# Autodesk Inventor assembly: 4in Omni Duallie
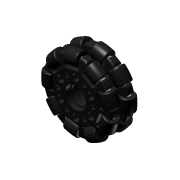
[picture p0: Inventor's stored thumbnail of the model, 180x180]
Saved by Autodesk Inventor 2011 (Build 150239000, 239)
## iProperties
Created: 2011-07-02
Part Number: 4in Omni Duallie
Document SubType Name: Assembly
Designer: Dan Niemitalo
Mass: 317.515 g
Surface Area: 1028.24 cm^2
Volume: 193.792 cm^3
Translation Standard: STEP AP203
FileName: //Amserv/amserver/AndyMark/Products/4 inch omni wheel/4 inch omni wheel dualie w 500 bearings.stp
PreProcessor: Unknown
PostProcessor: Build: 282, Release: 2011 SP1 - Date: Thu 08/05/2010
Sent Units: millimeter
Uncertainty: 0.001
Author: Dan Niemitalo
## Documents named in this file (3)
- H:\Nemo\Documents\Robotics\COTS Parts\Wheels\4in Omni Dualie.iam
- H:\Nemo\Documents\Robotics\Wheels and Sprockets\4 inch omni wheel no bearings.iam
- H:\Nemo\Documents\Robotics\COTS Parts\Sprockets\250 sprocket spacer.ipt
## Components (3 placed, 2 different names)
1. 250 sprocket spacer:1 — Mate:1, Mate:2, Mate:3, Mate:5, Mate:6, Mate:7
2. 4 inch omni wheel no bearings:1 [sub-assembly] — Mate:2, Mate:6, Mate:7
3. 4 inch omni wheel no bearings:2 [sub-assembly] — Mate:1, Mate:3, Mate:5
## Relationships (6: Mate 6)
- Mate:1: 250 sprocket spacer:1 ↔ 4 inch omni wheel no bearings:2
- Mate:2: 250 sprocket spacer:1 ↔ 4 inch omni wheel no bearings:1
- Mate:3: 250 sprocket spacer:1 ↔ 4 inch omni wheel no bearings:2
- Mate:5: 250 sprocket spacer:1 ↔ 4 inch omni wheel no bearings:2
- Mate:6: 250 sprocket spacer:1 ↔ 4 inch omni wheel no bearings:1
- Mate:7: 250 sprocket spacer:1 ↔ 4 inch omni wheel no bearings:1
